# Autodesk Inventor assembly: base_assambly
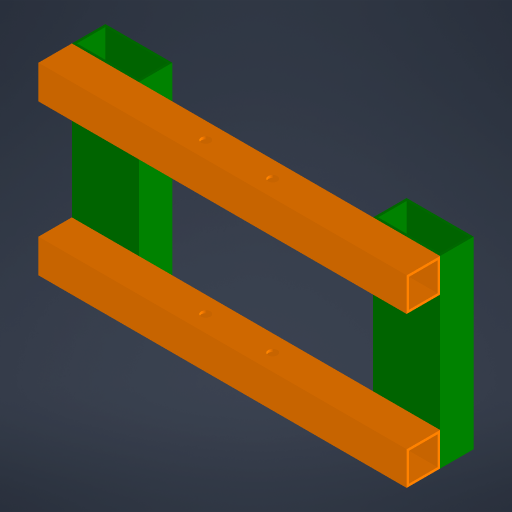
[picture p0: Inventor's stored thumbnail of the model, 512x512]
Saved by Autodesk Inventor 2024 (Build 280153000, 153)
## iProperties
Created: 2023-09-25
Part Number: base_assambly
Document SubType Name: Assembly
Designer: user
Author: user
## Documents named in this file (3)
- D:\Docs\Robot\3d_v2\base\base_assambly.iam
- D:\Docs\Robot\3d_v2\base\fb_axis.ipt
- D:\Docs\Robot\3d_v2\base\side_axis.ipt
## Components (4 placed, 2 different names)
1. fb_axis:1 — Совмещение:1, Совмещение:2, Совмещение:3, Заподлицо:3, Заподлицо:5, Совмещение:6
2. fb_axis:2 — Заподлицо:4, Заподлицо:6, Заподлицо:7, Заподлицо:8, Совмещение:4, Совмещение:5
3. side_axis:1 — Заподлицо:3, Заподлицо:4, Заподлицо:5, Заподлицо:8, Совмещение:5, Совмещение:6
4. side_axis:2 — Заподлицо:6, Заподлицо:7, Совмещение:4
## Relationships (12: Mate 6, Flush 6)
- Совмещение:1 [Mate]: fb_axis:1
- Совмещение:2 [Mate]: fb_axis:1
- Совмещение:3 [Mate]: fb_axis:1
- Заподлицо:3 [Flush]: fb_axis:1 ↔ side_axis:1
- Заподлицо:4 [Flush]: fb_axis:2 ↔ side_axis:1
- Заподлицо:5 [Flush]: fb_axis:1 ↔ side_axis:1
- Заподлицо:6 [Flush]: fb_axis:2 ↔ side_axis:2
- Заподлицо:7 [Flush]: fb_axis:2 ↔ side_axis:2
- Заподлицо:8 [Flush]: fb_axis:2 ↔ side_axis:1
- Совмещение:4 [Mate]: fb_axis:2 ↔ side_axis:2
- Совмещение:5 [Mate]: fb_axis:2 ↔ side_axis:1
- Совмещение:6 [Mate]: fb_axis:1 ↔ side_axis:1
